# Autodesk Inventor assembly: chain(c)
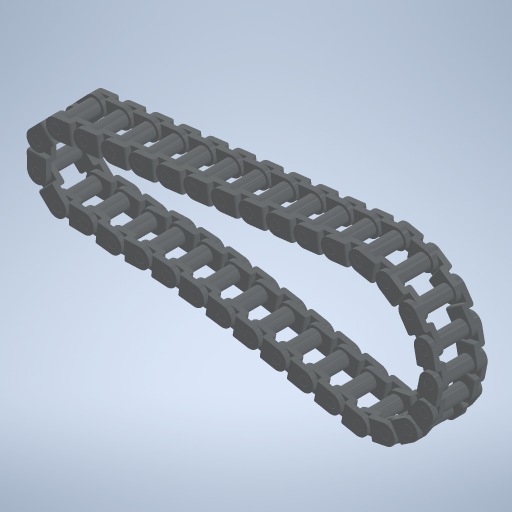
[picture p0: Inventor's stored thumbnail of the model, 512x512]
Saved by Autodesk Inventor 2023 (Build 270158000, 158)
## iProperties
Created: 2022-08-08
Part Number: chain(c)
Document SubType Name: Assembly
Designer: aaron
Author: aaron
## Documents named in this file (4)
- C:\Users\aaron\Documents\Inventor\Spin Up\library\Motion\New Sprockets\chain(c).iam
- C:\Users\aaron\Documents\Inventor\Spin Up\library\Motion\New Sprockets\8T.ipt
- C:\Users\aaron\Documents\Inventor\Spin Up\library\Motion\New Sprockets\16T.ipt
- C:\Users\aaron\Documents\Inventor\Spin Up\library\Motion\New Sprockets\IQ chain.ipt
## Components (35 placed, 3 different names)
1. 8T:1 — Mate:1, Mate:42, Mate:43, Mate:44, Mate:45
2. 16T:1 — Mate:1, Mate:33, Flush:32, Mate:34, Mate:35, Mate:36, Mate:37, Mate:38, Mate:39, Mate:40, Mate:41
3. IQ chain:1 — Mate:2, Flush:1, Mate:45, Mate:47
4. IQ chain:2 — Mate:2, Flush:1, Mate:4, Flush:3, Mate:44
5. IQ chain:3 — Mate:4, Flush:3, Mate:43
6. IQ chain:4 — Mate:8, Flush:7, Mate:42
7. IQ chain:5 — Mate:8, Flush:7
8. IQ chain:6
9. IQ chain:7
10. IQ chain:8 — Mate:16, Flush:15
11. IQ chain:9 — Mate:16, Flush:15
12. IQ chain:10
13. IQ chain:11
14. IQ chain:12
15. IQ chain:13
16. IQ chain:14
17. IQ chain:15 — Mate:33
18. IQ chain:16 — Mate:32, Flush:31, Flush:32, Mate:34
19. IQ chain:17 — Mate:32, Flush:31, Mate:35
20. IQ chain:18 — Mate:36
21. IQ chain:19 — Mate:37
22. IQ chain:20 — Mate:38
23. IQ chain:21 — Mate:39
24. IQ chain:22 — Mate:40
25. IQ chain:23 — Mate:41
26. IQ chain:24
27. IQ chain:25
28. IQ chain:26
29. IQ chain:27
30. IQ chain:28
31. IQ chain:29
32. IQ chain:30
33. IQ chain:31
34. IQ chain:32 — Mate:46, Flush:33
35. IQ chain:33 — Mate:46, Flush:33, Mate:47
## Relationships (80: Mate 47, Flush 33)
- Mate:1 (66.04 mm): 8T:1 ↔ 16T:1
- Mate:2: IQ chain:1 ↔ IQ chain:2
- Flush:1: IQ chain:1 ↔ IQ chain:2
- [Mate]: IQ chain:3 ↔ IQ chain:4
- [Flush]: IQ chain:3 ↔ IQ chain:4
- Mate:4: IQ chain:2 ↔ IQ chain:3
- Flush:3: IQ chain:2 ↔ IQ chain:3
- [Mate]: IQ chain:5 ↔ IQ chain:6
- [Flush]: IQ chain:5 ↔ IQ chain:6
- [Mate]: IQ chain:7 ↔ IQ chain:8
- [Flush]: IQ chain:7 ↔ IQ chain:8
- [Mate]: IQ chain:6 ↔ IQ chain:7
- [Flush]: IQ chain:6 ↔ IQ chain:7
- Mate:8: IQ chain:4 ↔ IQ chain:5
- Flush:7: IQ chain:4 ↔ IQ chain:5
- [Mate]: IQ chain:9 ↔ IQ chain:10
- [Flush]: IQ chain:9 ↔ IQ chain:10
- [Mate]: IQ chain:11 ↔ IQ chain:12
- [Flush]: IQ chain:11 ↔ IQ chain:12
- [Mate]: IQ chain:10 ↔ IQ chain:11
- [Flush]: IQ chain:10 ↔ IQ chain:11
- [Mate]: IQ chain:13 ↔ IQ chain:14
- [Flush]: IQ chain:13 ↔ IQ chain:14
- [Mate]: IQ chain:15 ↔ IQ chain:16
- [Flush]: IQ chain:15 ↔ IQ chain:16
- [Mate]: IQ chain:14 ↔ IQ chain:15
- [Flush]: IQ chain:14 ↔ IQ chain:15
- [Mate]: IQ chain:12 ↔ IQ chain:13
- [Flush]: IQ chain:12 ↔ IQ chain:13
- Mate:16: IQ chain:8 ↔ IQ chain:9
- Flush:15: IQ chain:8 ↔ IQ chain:9
- [Mate]: IQ chain:17 ↔ IQ chain:18
- [Flush]: IQ chain:17 ↔ IQ chain:18
- [Mate]: IQ chain:19 ↔ IQ chain:20
- [Flush]: IQ chain:19 ↔ IQ chain:20
- [Mate]: IQ chain:18 ↔ IQ chain:19
- [Flush]: IQ chain:18 ↔ IQ chain:19
- [Mate]: IQ chain:21 ↔ IQ chain:22
- [Flush]: IQ chain:21 ↔ IQ chain:22
- [Mate]: IQ chain:23 ↔ IQ chain:24
- [Flush]: IQ chain:23 ↔ IQ chain:24
- [Mate]: IQ chain:22 ↔ IQ chain:23
- [Flush]: IQ chain:22 ↔ IQ chain:23
- [Mate]: IQ chain:20 ↔ IQ chain:21
- [Flush]: IQ chain:20 ↔ IQ chain:21
- [Mate]: IQ chain:25 ↔ IQ chain:26
- [Flush]: IQ chain:25 ↔ IQ chain:26
- [Mate]: IQ chain:27 ↔ IQ chain:28
- [Flush]: IQ chain:27 ↔ IQ chain:28
- [Mate]: IQ chain:26 ↔ IQ chain:27
- [Flush]: IQ chain:26 ↔ IQ chain:27
- [Mate]: IQ chain:29 ↔ IQ chain:30
- [Flush]: IQ chain:29 ↔ IQ chain:30
- [Mate]: IQ chain:31 ↔ IQ chain:32
- [Flush]: IQ chain:31 ↔ IQ chain:32
- [Mate]: IQ chain:30 ↔ IQ chain:31
- [Flush]: IQ chain:30 ↔ IQ chain:31
- [Mate]: IQ chain:28 ↔ IQ chain:29
- [Flush]: IQ chain:28 ↔ IQ chain:29
- [Mate]: IQ chain:24 ↔ IQ chain:25
- [Flush]: IQ chain:24 ↔ IQ chain:25
- Mate:32: IQ chain:16 ↔ IQ chain:17
- Flush:31: IQ chain:16 ↔ IQ chain:17
- Mate:33: 16T:1 ↔ IQ chain:15
- Flush:32: 16T:1 ↔ IQ chain:16
- Mate:34: 16T:1 ↔ IQ chain:16
- Mate:35: 16T:1 ↔ IQ chain:17
- Mate:36: 16T:1 ↔ IQ chain:18
- Mate:37: 16T:1 ↔ IQ chain:19
- Mate:38: 16T:1 ↔ IQ chain:20
- Mate:39: 16T:1 ↔ IQ chain:21
- Mate:40: 16T:1 ↔ IQ chain:22
- Mate:41: 16T:1 ↔ IQ chain:23
- Mate:42: 8T:1 ↔ IQ chain:4
- Mate:43: 8T:1 ↔ IQ chain:3
- Mate:44: 8T:1 ↔ IQ chain:2
- Mate:45: 8T:1 ↔ IQ chain:1
- Mate:46: IQ chain:32 ↔ IQ chain:33
- Flush:33: IQ chain:32 ↔ IQ chain:33
- Mate:47: IQ chain:1 ↔ IQ chain:33
## Named parameters: d3_d2 = 0 mm, d4_d1 = 0 mm, d7_d2 = 0 mm, d8_d3_d2 = 0 mm, d9_d4_d1 = 0 mm, d10_d5 = 0 mm, d11_d6 = 0 mm, d12_d1 = 0 mm, d15_d2 = 0 mm, d16_d3_d2 = 0 mm, d17_d4_d1 = 0 mm, d18_d5 = 0 mm, d19_d6 = 0 mm, d20_d7_d2 = 0 mm, d21_d8_d3_d2 = 0 mm, d22_d9_d4_d1 = 0 mm, d23_d10_d5 = 0 mm, d24_d11_d6 = 0 mm, d25_d12_d1 = 0 mm, d26_d13 = 0 mm, d27_d14 = 0 mm, d28_d1 = 0 mm, d31_d2 = 0 mm, d32_d3_d2 = 0 mm, d33_d4_d1 = 0 mm, d34_d5 = 0 mm, d35_d6 = 0 mm, d36_d7_d2 = 0 mm, d37_d8_d3_d2 = 0 mm, d38_d9_d4_d1 = 0 mm, d39_d10_d5 = 0 mm, d40_d11_d6 = 0 mm, d41_d12_d1 = 0 mm, d42_d13 = 0 mm, d43_d14 = 0 mm, d44_d15_d2 = 0 mm, d45_d16_d3_d2 = 0 mm, d46_d17_d4_d1 = 0 mm, d47_d18_d5 = 0 mm, d48_d19_d6 = 0 mm, d49_d20_d7_d2 = 0 mm, d50_d21_d8_d3_d2 = 0 mm, d51_d22_d9_d4_d1 = 0 mm, d52_d23_d10_d5 = 0 mm, d53_d24_d11_d6 = 0 mm, d54_d25_d12_d1 = 0 mm, d55_d26_d13 = 0 mm, d56_d27_d14 = 0 mm, d57_d28_d1 = 0 mm, d58_d29 = 0 mm, d59_d30 = 0 mm, d60_d1 = 0 mm
